# Autodesk Inventor assembly: EnsamblajesJuntos
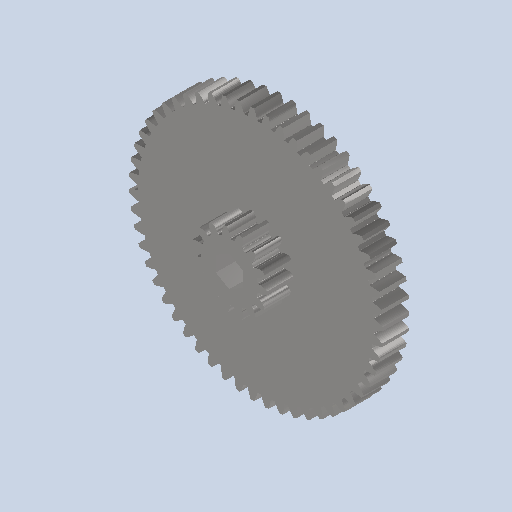
[picture p0: Inventor's stored thumbnail of the model, 512x512]
Saved by Autodesk Inventor 2022 (Build 260153000, 153)
## iProperties
Created: 2022-03-01
Part Number: EnsamblajesJuntos
Document SubType Name: Assembly
Designer: Marco
Author: Marco
## Documents named in this file (3)
- C:\Users\steff\Desktop\9noSemestre\Diseño\MiniProyecto\EnsamblajesJuntos.iam
- C:\Users\steff\Desktop\9noSemestre\Diseño\MiniProyecto\Engranaje.ipt
- C:\Users\steff\Desktop\9noSemestre\Diseño\MiniProyecto\Piñon.ipt
## Components (2 placed, 2 different names)
1. Engranaje:1 — Coincidencia:1, Coincidencia:2, Coincidencia:3
2. Piñon:1 — Coincidencia:1, Coincidencia:2, Coincidencia:3
## Relationships (3: Mate 3)
- Coincidencia:1 [Mate]: Engranaje:1 ↔ Piñon:1
- Coincidencia:2 [Mate]: Engranaje:1 ↔ Piñon:1
- Coincidencia:3 [Mate]: Engranaje:1 ↔ Piñon:1
